# Autodesk Inventor assembly: ARM_033_IntakeFULLAssembly
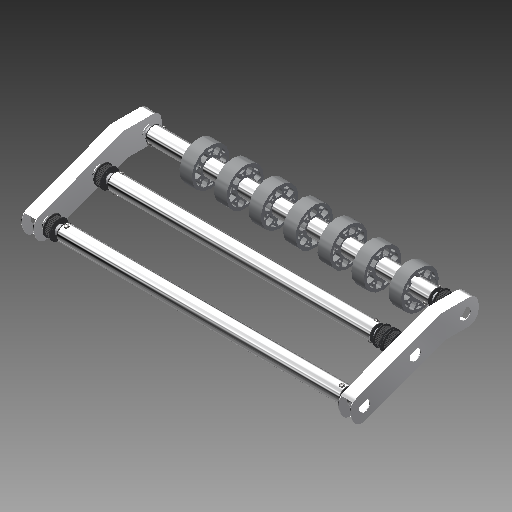
[picture p0: Inventor's stored thumbnail of the model, 512x512]
Saved by Autodesk Inventor 2018 (Build 220112000, 112)
## iProperties
Created: 2020-02-05
Part Number: ARM_033_IntakeFULLAssembly
Document SubType Name: Assembly
Designer: 22turnmaxw
Mass: 1974.13 g
Surface Area: 8383.72 cm^2
Volume: 1132.29 cm^3
Density: 1.74348 g/cm^3
Author: 22turnmaxw
## Documents named in this file (5)
- C:\Users\user\Documents\GrabCAD\New folder\Build season\ARM_033_IntakeFULLAssembly.iam
- C:\Users\user\Documents\GrabCAD\New folder\Build season\ARM_031_TwoPieceIntake.iam
- C:\Users\user\Documents\GrabCAD\New folder\Build season\ARM_032_3_OD_Straight_Flex_Wheel_217-6447.ipt
- C:\Users\user\Documents\GrabCAD\New folder\Build season\ARM_036_TopandBottomRollers.iam
- C:\Users\user\Documents\GrabCAD\New folder\Build season\ARM_039_MiddleRoller.iam
## Components (12 placed, 4 different names)
1. ARM_031_TwoPieceIntake:1 [sub-assembly] — Flush:1, Flush:2, Mate:1, Mate:36, Mate:37, Mate:40, Mate:41
2. ARM_031_TwoPieceIntake:2 [sub-assembly] — Flush:1, Flush:2, Mate:1, Mate:38, Mate:39
3. ARM_032_3_OD_Straight_Flex_Wheel_217-6447:1 — Mate:20, Mate:21, Rotation:13, Rotation:14
4. ARM_032_3_OD_Straight_Flex_Wheel_217-6447:2 — Mate:24, Rotation:16
5. ARM_032_3_OD_Straight_Flex_Wheel_217-6447:3 — Mate:22, Mate:23, Mate:24, Rotation:15, Rotation:16
6. ARM_032_3_OD_Straight_Flex_Wheel_217-6447:5 — Mate:18, Rotation:11
7. ARM_032_3_OD_Straight_Flex_Wheel_217-6447:6 — Mate:19, Mate:20, Rotation:12, Rotation:13
8. ARM_032_3_OD_Straight_Flex_Wheel_217-6447:7 — Mate:18, Mate:19, Rotation:11, Rotation:12
9. ARM_032_3_OD_Straight_Flex_Wheel_217-6447:8 — Mate:21, Mate:22, Mate:23, Rotation:14, Rotation:15
10. ARM_036_TopandBottomRollers:1 [sub-assembly] — Mate:38, Mate:39
11. ARM_036_TopandBottomRollers:2 [sub-assembly] — Mate:36, Mate:37
12. ARM_039_MiddleRoller:1 [sub-assembly] — Mate:40, Mate:41
## Relationships (22: Mate 14, RelateRotation 6, Flush 2)
- Flush:1: ARM_031_TwoPieceIntake:1 ↔ ARM_031_TwoPieceIntake:2
- Flush:2: ARM_031_TwoPieceIntake:1 ↔ ARM_031_TwoPieceIntake:2
- Mate:1 (615.95 mm): ARM_031_TwoPieceIntake:1 ↔ ARM_031_TwoPieceIntake:2
- Mate:18 (44.45 mm): ARM_032_3_OD_Straight_Flex_Wheel_217-6447:5 ↔ ARM_032_3_OD_Straight_Flex_Wheel_217-6447:7
- Mate:19 (44.45 mm): ARM_032_3_OD_Straight_Flex_Wheel_217-6447:6 ↔ ARM_032_3_OD_Straight_Flex_Wheel_217-6447:7
- Mate:20 (44.45 mm): ARM_032_3_OD_Straight_Flex_Wheel_217-6447:1 ↔ ARM_032_3_OD_Straight_Flex_Wheel_217-6447:6
- Mate:21 (44.45 mm): ARM_032_3_OD_Straight_Flex_Wheel_217-6447:1 ↔ ARM_032_3_OD_Straight_Flex_Wheel_217-6447:8
- Mate:22 (44.45 mm): ARM_032_3_OD_Straight_Flex_Wheel_217-6447:3 ↔ ARM_032_3_OD_Straight_Flex_Wheel_217-6447:8
- Mate:23 (44.45 mm): ARM_032_3_OD_Straight_Flex_Wheel_217-6447:3 ↔ ARM_032_3_OD_Straight_Flex_Wheel_217-6447:8
- Mate:24 (44.45 mm): ARM_032_3_OD_Straight_Flex_Wheel_217-6447:2 ↔ ARM_032_3_OD_Straight_Flex_Wheel_217-6447:3
- Rotation:11 [RelateRotation] (1 ul): ARM_032_3_OD_Straight_Flex_Wheel_217-6447:5 ↔ ARM_032_3_OD_Straight_Flex_Wheel_217-6447:7
- Rotation:12 [RelateRotation] (1 ul): ARM_032_3_OD_Straight_Flex_Wheel_217-6447:6 ↔ ARM_032_3_OD_Straight_Flex_Wheel_217-6447:7
- Rotation:13 [RelateRotation] (1 ul): ARM_032_3_OD_Straight_Flex_Wheel_217-6447:1 ↔ ARM_032_3_OD_Straight_Flex_Wheel_217-6447:6
- Rotation:14 [RelateRotation] (1 ul): ARM_032_3_OD_Straight_Flex_Wheel_217-6447:1 ↔ ARM_032_3_OD_Straight_Flex_Wheel_217-6447:8
- Rotation:15 [RelateRotation] (1 ul): ARM_032_3_OD_Straight_Flex_Wheel_217-6447:3 ↔ ARM_032_3_OD_Straight_Flex_Wheel_217-6447:8
- Rotation:16 [RelateRotation] (1 ul): ARM_032_3_OD_Straight_Flex_Wheel_217-6447:2 ↔ ARM_032_3_OD_Straight_Flex_Wheel_217-6447:3
- Mate:36: ARM_031_TwoPieceIntake:1 ↔ ARM_036_TopandBottomRollers:2
- Mate:37: ARM_031_TwoPieceIntake:1 ↔ ARM_036_TopandBottomRollers:2
- Mate:38: ARM_031_TwoPieceIntake:2 ↔ ARM_036_TopandBottomRollers:1
- Mate:39: ARM_031_TwoPieceIntake:2 ↔ ARM_036_TopandBottomRollers:1
- Mate:40: ARM_031_TwoPieceIntake:1 ↔ ARM_039_MiddleRoller:1
- Mate:41: ARM_031_TwoPieceIntake:1 ↔ ARM_039_MiddleRoller:1
